# Autodesk Inventor assembly: Middle layer
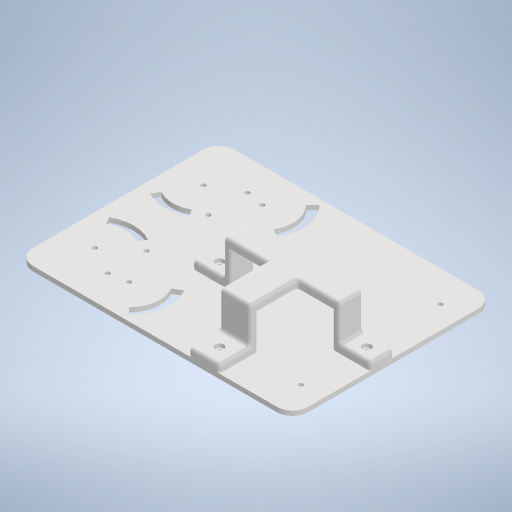
[picture p0: Inventor's stored thumbnail of the model, 512x512]
Saved by Autodesk Inventor 2023 (Build 270158000, 158)
## iProperties
Created: 2024-10-04
Part Number: Middle layer
Document SubType Name: Assembly
Designer: bw1293
Author: bw1293
## Documents named in this file (3)
- \\userfs\bw1293\w2k\Inventor\Bw RDAC 1\Middle layer.iam
- \\userfs\bw1293\w2k\Inventor\Bw RDAC 1\Middle layer.ipt
- \\userfs\bw1293\w2k\Inventor\Bw RDAC 1\Battery mount_MIR.ipt
## Components (2 placed, 2 different names)
1. Middle layer:1 — Mate:1
2. Battery mount_MIR:1 — Mate:1
## Relationships (1: Mate 1)
- Mate:1: Middle layer:1 ↔ Battery mount_MIR:1
